# Autodesk Inventor assembly: Drive Roller Assembly 2
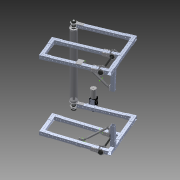
[picture p0: Inventor's stored thumbnail of the model, 180x180]
Saved by Autodesk Inventor 2014 (Build 180170000, 170)
## iProperties
Created: 2014-01-12
Part Number: Drive Roller Assembly 2
Document SubType Name: Assembly
Designer: Michael
Mass: 4500.32 g
Surface Area: 14923 cm^2
Volume: 1330.27 cm^3
Density: 3.383 g/cm^3
Author: Michael
## Documents named in this file (23)
- C:\Users\Michael\Documents\GitHub\2014buildCAD\New Collector\Drive Roller Assembly 2.iam
- C:\Users\Michael\Documents\GitHub\2014buildCAD\Collector\Hex Shaft Collar 1-2 in (7552K500).ipt
- C:\Users\Michael\Documents\GitHub\2014buildCAD\Collector\Roller End Cap Drive (3-D Printed).ipt
- C:\Users\Michael\Documents\GitHub\2014buildCAD\Collector\Vex Pro VersaPlanetary Side Mount.ipt
- C:\Users\Michael\Documents\GitHub\2014buildCAD\Collector\VersaPlanetary (Fixed).iam
- C:\Users\Michael\Documents\GitHub\2014buildCAD\New Collector\Polycarbonate Roller 2 OD 1-16 Thick (8585K64).ipt
- C:\Users\Michael\Documents\GitHub\2014buildCAD\New Collector\Hex Bearing 1-2 in (FR8ZZ-Hex, am-0279).ipt
- C:\Users\Michael\Documents\GitHub\2014buildCAD\New Collector\Hex Shaft Collar 1-2 in (7552K500).ipt
- C:\Users\Michael\Documents\GitHub\2014buildCAD\New Collector\Roller End Cap Drive (3-D Printed).ipt
- C:\Users\Michael\Documents\GitHub\2014buildCAD\New Collector\Vex Pro End Bearing Mount.ipt
- C:\Users\Michael\Documents\GitHub\2014buildCAD\New Collector\Vex Pro 1x1 rectangular tubing 14 in length.ipt
- C:\Users\Michael\Documents\GitHub\2014buildCAD\New Collector\Hex Shaft Aluminum 1-2 in (am-2291).ipt
- C:\Users\Michael\Documents\GitHub\2014buildCAD\New Collector\Timing Pulley (HTD 5mm) - 18T 9mm Double Flange, 1-2 in Hex (VexPro).ipt
- C:\Users\Michael\Documents\GitHub\2014buildCAD\New Collector\Clamp with Piston Assembly.iam
- C:\Users\Michael\Documents\GitHub\2014buildCAD\New Collector\Vex Pro 90 degree gusset.ipt
- C:\Users\Michael\Documents\GitHub\2014buildCAD\New Collector\Vex Pro 1x1 rectangular tubing 2 in length.ipt
- C:\Users\Michael\Documents\GitHub\2014buildCAD\New Collector\Hex Shaft 3-8 in (am-0855).ipt
- C:\Users\Michael\Documents\GitHub\2014buildCAD\New Collector\Hex Shaft Collar 3-8 in (7552K300).ipt
- C:\Users\Michael\Documents\GitHub\2014buildCAD\New Collector\3 Postion Pneumatic Cylinder (9-16 in Bore, .25 in,2 in stroke).iam
- C:\Users\Michael\Documents\GitHub\2014buildCAD\New Collector\Vex Pro 1x1 rectangular tubing 6 in length.ipt
- C:\Users\Michael\Documents\GitHub\2014buildCAD\New Collector\Pneumatic Piston Back Flange (Custom).ipt
- C:\Users\Michael\Documents\GitHub\2014buildCAD\New Collector\Pneumatic Piston Front Flange (Custom).ipt
- C:\Users\Michael\Documents\GitHub\2014buildCAD\New Collector\Pneumatic Piston Front Flange (Right Custom).ipt
## Components (61 placed, 20 different names)
1. Roller End Cap Drive (3-D Printed):2 — Mate:154, Mate:155, Mate:156, Mate:157, Mate:158
2. Vex Pro VersaPlanetary Side Mount:1 — Insert:29, Insert:30, Mate:136, Mate:181, Mate:182
3. VersaPlanetary (Fixed):1 [sub-assembly] — Insert:29, Insert:30, Mate:113, Mate:114, Mate:120, Mate:121, Mate:153
4. Hex Shaft Collar 1-2 in (7552K500):9 — Mate:113, Mate:114
5. Hex Shaft Collar 1-2 in (7552K500):10 — Mate:120, Mate:121
6. Polycarbonate Roller 2 OD 1-16 Thick (8585K64):3 — Mate:157, Mate:158, Mate:159, Mate:160
7. Hex Bearing 1-2 in (FR8ZZ-Hex, am-0279):3 — Mate:128, Mate:129, Mate:134, Mate:156
8. Roller End Cap Drive (3-D Printed):5 — Mate:159, Mate:160, Mate:174
9. Vex Pro 1x1 rectangular tubing 14 in length:2 — Mate:122, Mate:123, Mate:124, Mate:125, Mate:126, Mate:127, Mate:136, Mate:181, Mate:182, Mate:198, Mate:199, Mate:200, Flush:9
10. Hex Shaft Aluminum 1-2 in (am-2291):1 — Flush:1, Mate:132, Mate:133, Mate:134, Mate:143, Mate:144, Mate:146, Mate:147, Mate:154, Mate:155, Mate:172, Mate:173, Mate:175, Mate:176, Mate:179, Mate:180
11. Vex Pro End Bearing Mount:4 — Mate:122, Mate:123, Mate:126, Mate:130, Mate:131
12. Vex Pro End Bearing Mount:5 — Mate:124, Mate:125, Mate:127, Mate:128, Mate:129
13. Hex Bearing 1-2 in (FR8ZZ-Hex, am-0279):4 — Mate:130, Mate:131, Flush:1, Mate:132, Mate:133, Mate:161
14. Timing Pulley (HTD 5mm) - 18T 9mm Double Flange, 1-2 in Hex (VexPro):3 — Mate:143, Mate:144, Mate:145, Mate:161
15. Hex Shaft Collar 1-2 in (7552K500):13 — Mate:145, Mate:146, Mate:147, Flush:2
16. Hex Shaft Collar 1-2 in (7552K500):14 — Flush:4, Mate:152
17. Timing Pulley (HTD 5mm) - 18T 9mm Double Flange, 1-2 in Hex (VexPro):4 — Mate:150, Flush:3, Mate:151, Flush:4, Mate:152
18. Hex Shaft Collar 1-2 in (7552K500):15 — Flush:2, Mate:150, Flush:3, Mate:151, Mate:153
19. Hex Bearing 1-2 in (FR8ZZ-Hex, am-0279):5 — Mate:178
20. Vex Pro 1x1 rectangular tubing 14 in length:3 — Mate:183, Mate:184, Mate:185, Mate:186, Mate:187, Mate:188, Flush:9
21. Vex Pro End Bearing Mount:7
22. Vex Pro End Bearing Mount:8
23. Hex Bearing 1-2 in (FR8ZZ-Hex, am-0279):6 — Mate:172, Mate:173, Mate:177
24. Hex Shaft Collar 1-2 in (7552K500):16 — Mate:178, Mate:179, Mate:180
25. Hex Shaft Collar 1-2 in (7552K500):17 — Mate:174, Mate:175, Mate:176, Mate:177
26. Clamp with Piston Assembly:1 [sub-assembly] — Mate:226, Mate:227, Flush:6, Mate:230, Mate:233, Mate:285, Mate:286, Mate:287
27. Vex Pro 1x1 rectangular tubing 14 in length:5 — Mate:189, Mate:190, Mate:191, Mate:203, Mate:210, Mate:211, Mate:221, Mate:222, Mate:223, Mate:264, Mate:265, Mate:266, Mate:267, Mate:268, Mate:269, Mate:270, Mate:272, Mate:273
28. Vex Pro 90 degree gusset:1 — Mate:186, Mate:187, Mate:188
29. Vex Pro 90 degree gusset:3 — Mate:183, Mate:184, Mate:185, Mate:189, Mate:190, Mate:191
30. Vex Pro 1x1 rectangular tubing 14 in length:6 — Mate:195, Mate:196, Mate:197, Mate:258, Mate:259, Mate:260, Mate:261, Mate:262, Mate:263, Mate:298, Mate:299, Mate:300, Mate:301, Mate:305, Mate:306
31. Vex Pro 90 degree gusset:5 — Mate:195, Mate:196, Mate:197, Mate:198, Mate:199, Mate:200
32. Vex Pro 90 degree gusset:6
33. Vex Pro 90 degree gusset:8 — Mate:203, Mate:210, Mate:211, Mate:212, Mate:213, Mate:214
34. Vex Pro 1x1 rectangular tubing 2 in length:1 — Mate:212, Mate:213, Mate:214
35. Vex Pro 90 degree gusset:10 — Mate:221, Mate:222, Mate:223
36. Vex Pro 1x1 rectangular tubing 2 in length:2 — Mate:224, Mate:225, Flush:5, Mate:271
37. Hex Shaft 3-8 in (am-0855):1 — Mate:224, Mate:225, Flush:5, Mate:226, Mate:227, Flush:6, Mate:228, Mate:229, Mate:231, Mate:232
38. Hex Shaft Collar 3-8 in (7552K300):1 — Mate:228, Mate:229, Mate:230
39. Hex Shaft Collar 3-8 in (7552K300):2 — Mate:231, Mate:232, Mate:233
40. Clamp with Piston Assembly:2 [sub-assembly] — Mate:311, Mate:312, Mate:313
41. Vex Pro 90 degree gusset:11 — Mate:253, Mate:254, Mate:255
42. Vex Pro 90 degree gusset:12 — Mate:261, Mate:262, Mate:263
43. Vex Pro 1x1 rectangular tubing 2 in length:3 — Mate:253, Mate:254, Mate:255
44. Vex Pro 90 degree gusset:13 — Mate:258, Mate:259, Mate:260
45. Vex Pro 1x1 rectangular tubing 2 in length:4
46. Hex Shaft 3-8 in (am-0855):2
47. Hex Shaft Collar 3-8 in (7552K300):3
48. Hex Shaft Collar 3-8 in (7552K300):4
49. 3 Postion Pneumatic Cylinder (9-16 in Bore, .25 in,2 in stroke):1 [sub-assembly] — Mate:280, Mate:281, Mate:282, Mate:288
50. Vex Pro 1x1 rectangular tubing 6 in length:1 — Mate:274, Mate:275, Mate:276, Mate:277, Mate:278, Mate:279
51. Vex Pro 90 degree gusset:14 — Mate:264, Mate:265, Mate:266, Mate:274, Mate:275, Mate:276
52. Vex Pro 90 degree gusset:15 — Mate:267, Mate:268, Mate:269
53. Vex Pro 90 degree gusset:16 — Mate:270, Mate:271, Mate:272, Mate:273
54. Pneumatic Piston Back Flange (Custom):1 — Mate:277, Mate:278, Mate:279, Mate:280, Mate:281, Mate:282
55. Pneumatic Piston Front Flange (Custom):1 — Mate:285, Mate:286, Mate:287, Mate:288
56. 3 Postion Pneumatic Cylinder (9-16 in Bore, .25 in,2 in stroke):2 [sub-assembly] — Mate:314
57. Vex Pro 1x1 rectangular tubing 6 in length:2 — Mate:302, Mate:303, Mate:304, Mate:307, Mate:308
58. Vex Pro 90 degree gusset:17 — Mate:300, Mate:301, Mate:305, Mate:306
59. Vex Pro 90 degree gusset:18 — Mate:298, Mate:299, Mate:302, Mate:303, Mate:304
60. Pneumatic Piston Back Flange (Custom):2 — Mate:307, Mate:308
61. Pneumatic Piston Front Flange (Right Custom):1 — Mate:311, Mate:312, Mate:313, Mate:314
## Relationships (177: Mate 166, Flush 9, Insert 2)
- Insert:29: Vex Pro VersaPlanetary Side Mount:1 ↔ VersaPlanetary (Fixed):1
- Insert:30: Vex Pro VersaPlanetary Side Mount:1 ↔ VersaPlanetary (Fixed):1
- Mate:113: VersaPlanetary (Fixed):1 ↔ Hex Shaft Collar 1-2 in (7552K500):9
- Mate:114: VersaPlanetary (Fixed):1 ↔ Hex Shaft Collar 1-2 in (7552K500):9
- Mate:120: VersaPlanetary (Fixed):1 ↔ Hex Shaft Collar 1-2 in (7552K500):10
- Mate:121: VersaPlanetary (Fixed):1 ↔ Hex Shaft Collar 1-2 in (7552K500):10
- Mate:122: Vex Pro 1x1 rectangular tubing 14 in length:2 ↔ Vex Pro End Bearing Mount:4
- Mate:123: Vex Pro 1x1 rectangular tubing 14 in length:2 ↔ Vex Pro End Bearing Mount:4
- Mate:124: Vex Pro 1x1 rectangular tubing 14 in length:2 ↔ Vex Pro End Bearing Mount:5
- Mate:125: Vex Pro 1x1 rectangular tubing 14 in length:2 ↔ Vex Pro End Bearing Mount:5
- Mate:126: Vex Pro 1x1 rectangular tubing 14 in length:2 ↔ Vex Pro End Bearing Mount:4
- Mate:127: Vex Pro 1x1 rectangular tubing 14 in length:2 ↔ Vex Pro End Bearing Mount:5
- Mate:128: Hex Bearing 1-2 in (FR8ZZ-Hex, am-0279):3 ↔ Vex Pro End Bearing Mount:5
- Mate:129: Hex Bearing 1-2 in (FR8ZZ-Hex, am-0279):3 ↔ Vex Pro End Bearing Mount:5
- Mate:130: Vex Pro End Bearing Mount:4 ↔ Hex Bearing 1-2 in (FR8ZZ-Hex, am-0279):4
- Mate:131: Vex Pro End Bearing Mount:4 ↔ Hex Bearing 1-2 in (FR8ZZ-Hex, am-0279):4
- Flush:1 (-25.4 mm): Hex Shaft Aluminum 1-2 in (am-2291):1 ↔ Hex Bearing 1-2 in (FR8ZZ-Hex, am-0279):4
- Mate:132: Hex Shaft Aluminum 1-2 in (am-2291):1 ↔ Hex Bearing 1-2 in (FR8ZZ-Hex, am-0279):4
- Mate:133: Hex Shaft Aluminum 1-2 in (am-2291):1 ↔ Hex Bearing 1-2 in (FR8ZZ-Hex, am-0279):4
- Mate:134: Hex Bearing 1-2 in (FR8ZZ-Hex, am-0279):3 ↔ Hex Shaft Aluminum 1-2 in (am-2291):1
- Mate:136: Vex Pro VersaPlanetary Side Mount:1 ↔ Vex Pro 1x1 rectangular tubing 14 in length:2
- Mate:143: Hex Shaft Aluminum 1-2 in (am-2291):1 ↔ Timing Pulley (HTD 5mm) - 18T 9mm Double Flange, 1-2 in Hex (VexPro):3
- Mate:144: Hex Shaft Aluminum 1-2 in (am-2291):1 ↔ Timing Pulley (HTD 5mm) - 18T 9mm Double Flange, 1-2 in Hex (VexPro):3
- Mate:145: Timing Pulley (HTD 5mm) - 18T 9mm Double Flange, 1-2 in Hex (VexPro):3 ↔ Hex Shaft Collar 1-2 in (7552K500):13
- Mate:146: Hex Shaft Aluminum 1-2 in (am-2291):1 ↔ Hex Shaft Collar 1-2 in (7552K500):13
- Mate:147: Hex Shaft Aluminum 1-2 in (am-2291):1 ↔ Hex Shaft Collar 1-2 in (7552K500):13
- [Mate]: Hex Shaft Collar 1-2 in (7552K500):14 ↔ Timing Pulley (HTD 5mm) - 18T 9mm Double Flange, 1-2 in Hex (VexPro):4
- [Mate]: Timing Pulley (HTD 5mm) - 18T 9mm Double Flange, 1-2 in Hex (VexPro):4 ↔ Hex Shaft Collar 1-2 in (7552K500):15
- Flush:2: Hex Shaft Collar 1-2 in (7552K500):13 ↔ Hex Shaft Collar 1-2 in (7552K500):15
- Mate:150: Timing Pulley (HTD 5mm) - 18T 9mm Double Flange, 1-2 in Hex (VexPro):4 ↔ Hex Shaft Collar 1-2 in (7552K500):15
- Flush:3: Timing Pulley (HTD 5mm) - 18T 9mm Double Flange, 1-2 in Hex (VexPro):4 ↔ Hex Shaft Collar 1-2 in (7552K500):15
- Mate:151: Timing Pulley (HTD 5mm) - 18T 9mm Double Flange, 1-2 in Hex (VexPro):4 ↔ Hex Shaft Collar 1-2 in (7552K500):15
- Flush:4: Hex Shaft Collar 1-2 in (7552K500):14 ↔ Timing Pulley (HTD 5mm) - 18T 9mm Double Flange, 1-2 in Hex (VexPro):4
- Mate:152: Hex Shaft Collar 1-2 in (7552K500):14 ↔ Timing Pulley (HTD 5mm) - 18T 9mm Double Flange, 1-2 in Hex (VexPro):4
- Mate:153: VersaPlanetary (Fixed):1 ↔ Hex Shaft Collar 1-2 in (7552K500):15
- Mate:154: Roller End Cap Drive (3-D Printed):2 ↔ Hex Shaft Aluminum 1-2 in (am-2291):1
- Mate:155: Roller End Cap Drive (3-D Printed):2 ↔ Hex Shaft Aluminum 1-2 in (am-2291):1
- Mate:156: Roller End Cap Drive (3-D Printed):2 ↔ Hex Bearing 1-2 in (FR8ZZ-Hex, am-0279):3
- Mate:157: Roller End Cap Drive (3-D Printed):2 ↔ Polycarbonate Roller 2 OD 1-16 Thick (8585K64):3
- Mate:158: Roller End Cap Drive (3-D Printed):2 ↔ Polycarbonate Roller 2 OD 1-16 Thick (8585K64):3
- Mate:159: Polycarbonate Roller 2 OD 1-16 Thick (8585K64):3 ↔ Roller End Cap Drive (3-D Printed):5
- Mate:160: Polycarbonate Roller 2 OD 1-16 Thick (8585K64):3 ↔ Roller End Cap Drive (3-D Printed):5
- Mate:161: Hex Bearing 1-2 in (FR8ZZ-Hex, am-0279):4 ↔ Timing Pulley (HTD 5mm) - 18T 9mm Double Flange, 1-2 in Hex (VexPro):3
- [Mate]: Vex Pro 1x1 rectangular tubing 14 in length:3 ↔ Vex Pro End Bearing Mount:7
- [Mate]: Vex Pro 1x1 rectangular tubing 14 in length:3 ↔ Vex Pro End Bearing Mount:7
- [Mate]: Vex Pro 1x1 rectangular tubing 14 in length:3 ↔ Vex Pro End Bearing Mount:8
- [Mate]: Vex Pro 1x1 rectangular tubing 14 in length:3 ↔ Vex Pro End Bearing Mount:8
- [Mate]: Vex Pro 1x1 rectangular tubing 14 in length:3 ↔ Vex Pro End Bearing Mount:7
- [Mate]: Vex Pro 1x1 rectangular tubing 14 in length:3 ↔ Vex Pro End Bearing Mount:8
- [Mate]: Hex Bearing 1-2 in (FR8ZZ-Hex, am-0279):5 ↔ Vex Pro End Bearing Mount:8
- [Mate]: Hex Bearing 1-2 in (FR8ZZ-Hex, am-0279):5 ↔ Vex Pro End Bearing Mount:8
- [Mate]: Vex Pro End Bearing Mount:7 ↔ Hex Bearing 1-2 in (FR8ZZ-Hex, am-0279):6
- [Mate]: Vex Pro End Bearing Mount:7 ↔ Hex Bearing 1-2 in (FR8ZZ-Hex, am-0279):6
- Mate:172: Hex Shaft Aluminum 1-2 in (am-2291):1 ↔ Hex Bearing 1-2 in (FR8ZZ-Hex, am-0279):6
- Mate:173: Hex Shaft Aluminum 1-2 in (am-2291):1 ↔ Hex Bearing 1-2 in (FR8ZZ-Hex, am-0279):6
- Mate:174: Roller End Cap Drive (3-D Printed):5 ↔ Hex Shaft Collar 1-2 in (7552K500):17
- Mate:175: Hex Shaft Aluminum 1-2 in (am-2291):1 ↔ Hex Shaft Collar 1-2 in (7552K500):17
- Mate:176: Hex Shaft Aluminum 1-2 in (am-2291):1 ↔ Hex Shaft Collar 1-2 in (7552K500):17
- Mate:177: Hex Bearing 1-2 in (FR8ZZ-Hex, am-0279):6 ↔ Hex Shaft Collar 1-2 in (7552K500):17
- Mate:178: Hex Bearing 1-2 in (FR8ZZ-Hex, am-0279):5 ↔ Hex Shaft Collar 1-2 in (7552K500):16
- Mate:179: Hex Shaft Aluminum 1-2 in (am-2291):1 ↔ Hex Shaft Collar 1-2 in (7552K500):16
- Mate:180: Hex Shaft Aluminum 1-2 in (am-2291):1 ↔ Hex Shaft Collar 1-2 in (7552K500):16
- Mate:181: Vex Pro VersaPlanetary Side Mount:1 ↔ Vex Pro 1x1 rectangular tubing 14 in length:2
- Mate:182: Vex Pro VersaPlanetary Side Mount:1 ↔ Vex Pro 1x1 rectangular tubing 14 in length:2
- Mate:183: Vex Pro 1x1 rectangular tubing 14 in length:3 ↔ Vex Pro 90 degree gusset:3
- Mate:184: Vex Pro 1x1 rectangular tubing 14 in length:3 ↔ Vex Pro 90 degree gusset:3
- Mate:185: Vex Pro 1x1 rectangular tubing 14 in length:3 ↔ Vex Pro 90 degree gusset:3
- Mate:186: Vex Pro 1x1 rectangular tubing 14 in length:3 ↔ Vex Pro 90 degree gusset:1
- Mate:187: Vex Pro 1x1 rectangular tubing 14 in length:3 ↔ Vex Pro 90 degree gusset:1
- Mate:188: Vex Pro 1x1 rectangular tubing 14 in length:3 ↔ Vex Pro 90 degree gusset:1
- Mate:189: Vex Pro 1x1 rectangular tubing 14 in length:5 ↔ Vex Pro 90 degree gusset:3
- Mate:190: Vex Pro 1x1 rectangular tubing 14 in length:5 ↔ Vex Pro 90 degree gusset:3
- Mate:191: Vex Pro 1x1 rectangular tubing 14 in length:5 ↔ Vex Pro 90 degree gusset:3
- [Mate]: Vex Pro 1x1 rectangular tubing 14 in length:6 ↔ Vex Pro 90 degree gusset:6
- [Mate]: Vex Pro 1x1 rectangular tubing 14 in length:6 ↔ Vex Pro 90 degree gusset:6
- [Mate]: Vex Pro 1x1 rectangular tubing 14 in length:6 ↔ Vex Pro 90 degree gusset:6
- Mate:195: Vex Pro 1x1 rectangular tubing 14 in length:6 ↔ Vex Pro 90 degree gusset:5
- Mate:196: Vex Pro 1x1 rectangular tubing 14 in length:6 ↔ Vex Pro 90 degree gusset:5
- Mate:197: Vex Pro 1x1 rectangular tubing 14 in length:6 ↔ Vex Pro 90 degree gusset:5
- Mate:198: Vex Pro 1x1 rectangular tubing 14 in length:2 ↔ Vex Pro 90 degree gusset:5
- Mate:199: Vex Pro 1x1 rectangular tubing 14 in length:2 ↔ Vex Pro 90 degree gusset:5
- Mate:200: Vex Pro 1x1 rectangular tubing 14 in length:2 ↔ Vex Pro 90 degree gusset:5
- Mate:203: Vex Pro 1x1 rectangular tubing 14 in length:5 ↔ Vex Pro 90 degree gusset:8
- Mate:210: Vex Pro 1x1 rectangular tubing 14 in length:5 ↔ Vex Pro 90 degree gusset:8
- Mate:211: Vex Pro 1x1 rectangular tubing 14 in length:5 ↔ Vex Pro 90 degree gusset:8
- Mate:212: Vex Pro 90 degree gusset:8 ↔ Vex Pro 1x1 rectangular tubing 2 in length:1
- Mate:213: Vex Pro 90 degree gusset:8 ↔ Vex Pro 1x1 rectangular tubing 2 in length:1
- Mate:214: Vex Pro 90 degree gusset:8 ↔ Vex Pro 1x1 rectangular tubing 2 in length:1
- [Mate]: Vex Pro 90 degree gusset:10 ↔ Vex Pro 1x1 rectangular tubing 2 in length:2
- [Mate]: Vex Pro 90 degree gusset:10 ↔ Vex Pro 1x1 rectangular tubing 2 in length:2
- [Mate]: Vex Pro 90 degree gusset:10 ↔ Vex Pro 1x1 rectangular tubing 2 in length:2
- Mate:221: Vex Pro 1x1 rectangular tubing 14 in length:5 ↔ Vex Pro 90 degree gusset:10
- Mate:222: Vex Pro 1x1 rectangular tubing 14 in length:5 ↔ Vex Pro 90 degree gusset:10
- Mate:223: Vex Pro 1x1 rectangular tubing 14 in length:5 ↔ Vex Pro 90 degree gusset:10
- Mate:224: Vex Pro 1x1 rectangular tubing 2 in length:2 ↔ Hex Shaft 3-8 in (am-0855):1
- Mate:225: Vex Pro 1x1 rectangular tubing 2 in length:2 ↔ Hex Shaft 3-8 in (am-0855):1
- Flush:5 (-19.05 mm): Vex Pro 1x1 rectangular tubing 2 in length:2 ↔ Hex Shaft 3-8 in (am-0855):1
- Mate:226: Clamp with Piston Assembly:1 ↔ Hex Shaft 3-8 in (am-0855):1
- Mate:227: Clamp with Piston Assembly:1 ↔ Hex Shaft 3-8 in (am-0855):1
- Flush:6 (-9.525 mm): Clamp with Piston Assembly:1 ↔ Hex Shaft 3-8 in (am-0855):1
- Mate:228: Hex Shaft 3-8 in (am-0855):1 ↔ Hex Shaft Collar 3-8 in (7552K300):1
- Mate:229: Hex Shaft 3-8 in (am-0855):1 ↔ Hex Shaft Collar 3-8 in (7552K300):1
- Mate:230: Clamp with Piston Assembly:1 ↔ Hex Shaft Collar 3-8 in (7552K300):1
- Mate:231: Hex Shaft 3-8 in (am-0855):1 ↔ Hex Shaft Collar 3-8 in (7552K300):2
- Mate:232: Hex Shaft 3-8 in (am-0855):1 ↔ Hex Shaft Collar 3-8 in (7552K300):2
- Mate:233: Clamp with Piston Assembly:1 ↔ Hex Shaft Collar 3-8 in (7552K300):2
- [Mate]: Vex Pro 90 degree gusset:12 ↔ Vex Pro 1x1 rectangular tubing 2 in length:3
- [Mate]: Vex Pro 90 degree gusset:12 ↔ Vex Pro 1x1 rectangular tubing 2 in length:3
- [Mate]: Vex Pro 90 degree gusset:12 ↔ Vex Pro 1x1 rectangular tubing 2 in length:3
- [Mate]: Vex Pro 90 degree gusset:13 ↔ Vex Pro 1x1 rectangular tubing 2 in length:4
- [Mate]: Vex Pro 90 degree gusset:13 ↔ Vex Pro 1x1 rectangular tubing 2 in length:4
- [Mate]: Vex Pro 90 degree gusset:13 ↔ Vex Pro 1x1 rectangular tubing 2 in length:4
- [Mate]: Vex Pro 1x1 rectangular tubing 2 in length:4 ↔ Hex Shaft 3-8 in (am-0855):2
- [Mate]: Vex Pro 1x1 rectangular tubing 2 in length:4 ↔ Hex Shaft 3-8 in (am-0855):2
- [Flush] (-19.05 mm): Vex Pro 1x1 rectangular tubing 2 in length:4 ↔ Hex Shaft 3-8 in (am-0855):2
- [Mate]: Clamp with Piston Assembly:2 ↔ Hex Shaft 3-8 in (am-0855):2
- [Mate]: Clamp with Piston Assembly:2 ↔ Hex Shaft 3-8 in (am-0855):2
- [Flush] (-9.525 mm): Clamp with Piston Assembly:2 ↔ Hex Shaft 3-8 in (am-0855):2
- [Mate]: Hex Shaft 3-8 in (am-0855):2 ↔ Hex Shaft Collar 3-8 in (7552K300):3
- [Mate]: Hex Shaft 3-8 in (am-0855):2 ↔ Hex Shaft Collar 3-8 in (7552K300):3
- [Mate]: Clamp with Piston Assembly:2 ↔ Hex Shaft Collar 3-8 in (7552K300):3
- [Mate]: Hex Shaft 3-8 in (am-0855):2 ↔ Hex Shaft Collar 3-8 in (7552K300):4
- [Mate]: Hex Shaft 3-8 in (am-0855):2 ↔ Hex Shaft Collar 3-8 in (7552K300):4
- [Mate]: Clamp with Piston Assembly:2 ↔ Hex Shaft Collar 3-8 in (7552K300):4
- Mate:253: Vex Pro 90 degree gusset:11 ↔ Vex Pro 1x1 rectangular tubing 2 in length:3
- Mate:254: Vex Pro 90 degree gusset:11 ↔ Vex Pro 1x1 rectangular tubing 2 in length:3
- Mate:255: Vex Pro 90 degree gusset:11 ↔ Vex Pro 1x1 rectangular tubing 2 in length:3
- Mate:258: Vex Pro 1x1 rectangular tubing 14 in length:6 ↔ Vex Pro 90 degree gusset:13
- Mate:259: Vex Pro 1x1 rectangular tubing 14 in length:6 ↔ Vex Pro 90 degree gusset:13
- Mate:260: Vex Pro 1x1 rectangular tubing 14 in length:6 ↔ Vex Pro 90 degree gusset:13
- Mate:261: Vex Pro 1x1 rectangular tubing 14 in length:6 ↔ Vex Pro 90 degree gusset:12
- Mate:262: Vex Pro 1x1 rectangular tubing 14 in length:6 ↔ Vex Pro 90 degree gusset:12
- Mate:263: Vex Pro 1x1 rectangular tubing 14 in length:6 ↔ Vex Pro 90 degree gusset:12
- Flush:9: Vex Pro 1x1 rectangular tubing 14 in length:2 ↔ Vex Pro 1x1 rectangular tubing 14 in length:3
- Mate:264: Vex Pro 1x1 rectangular tubing 14 in length:5 ↔ Vex Pro 90 degree gusset:14
- Mate:265: Vex Pro 1x1 rectangular tubing 14 in length:5 ↔ Vex Pro 90 degree gusset:14
- Mate:266: Vex Pro 1x1 rectangular tubing 14 in length:5 ↔ Vex Pro 90 degree gusset:14
- Mate:267: Vex Pro 1x1 rectangular tubing 14 in length:5 ↔ Vex Pro 90 degree gusset:15
- Mate:268: Vex Pro 1x1 rectangular tubing 14 in length:5 ↔ Vex Pro 90 degree gusset:15
- Mate:269: Vex Pro 1x1 rectangular tubing 14 in length:5 ↔ Vex Pro 90 degree gusset:15
- Mate:270: Vex Pro 1x1 rectangular tubing 14 in length:5 ↔ Vex Pro 90 degree gusset:16
- Mate:271: Vex Pro 1x1 rectangular tubing 2 in length:2 ↔ Vex Pro 90 degree gusset:16
- Mate:272: Vex Pro 1x1 rectangular tubing 14 in length:5 ↔ Vex Pro 90 degree gusset:16
- Mate:273: Vex Pro 1x1 rectangular tubing 14 in length:5 ↔ Vex Pro 90 degree gusset:16
- Mate:274: Vex Pro 1x1 rectangular tubing 6 in length:1 ↔ Vex Pro 90 degree gusset:14
- Mate:275: Vex Pro 1x1 rectangular tubing 6 in length:1 ↔ Vex Pro 90 degree gusset:14
- Mate:276: Vex Pro 1x1 rectangular tubing 6 in length:1 ↔ Vex Pro 90 degree gusset:14
- Mate:277: Vex Pro 1x1 rectangular tubing 6 in length:1 ↔ Pneumatic Piston Back Flange (Custom):1
- Mate:278: Vex Pro 1x1 rectangular tubing 6 in length:1 ↔ Pneumatic Piston Back Flange (Custom):1
- Mate:279: Vex Pro 1x1 rectangular tubing 6 in length:1 ↔ Pneumatic Piston Back Flange (Custom):1
- Mate:280: 3 Postion Pneumatic Cylinder (9-16 in Bore, .25 in,2 in stroke):1 ↔ Pneumatic Piston Back Flange (Custom):1
- Mate:281: 3 Postion Pneumatic Cylinder (9-16 in Bore, .25 in,2 in stroke):1 ↔ Pneumatic Piston Back Flange (Custom):1
- Mate:282: 3 Postion Pneumatic Cylinder (9-16 in Bore, .25 in,2 in stroke):1 ↔ Pneumatic Piston Back Flange (Custom):1
- Mate:285: Clamp with Piston Assembly:1 ↔ Pneumatic Piston Front Flange (Custom):1
- Mate:286: Clamp with Piston Assembly:1 ↔ Pneumatic Piston Front Flange (Custom):1
- Mate:287: Clamp with Piston Assembly:1 ↔ Pneumatic Piston Front Flange (Custom):1
- Mate:288: 3 Postion Pneumatic Cylinder (9-16 in Bore, .25 in,2 in stroke):1 ↔ Pneumatic Piston Front Flange (Custom):1
- [Mate]: Vex Pro 1x1 rectangular tubing 6 in length:2 ↔ Vex Pro 90 degree gusset:17
- [Mate]: Vex Pro 1x1 rectangular tubing 6 in length:2 ↔ Pneumatic Piston Back Flange (Custom):2
- [Mate]: 3 Postion Pneumatic Cylinder (9-16 in Bore, .25 in,2 in stroke):2 ↔ Pneumatic Piston Back Flange (Custom):2
- [Mate]: 3 Postion Pneumatic Cylinder (9-16 in Bore, .25 in,2 in stroke):2 ↔ Pneumatic Piston Back Flange (Custom):2
- [Mate]: 3 Postion Pneumatic Cylinder (9-16 in Bore, .25 in,2 in stroke):2 ↔ Pneumatic Piston Back Flange (Custom):2
- Mate:298: Vex Pro 1x1 rectangular tubing 14 in length:6 ↔ Vex Pro 90 degree gusset:18
- Mate:299: Vex Pro 1x1 rectangular tubing 14 in length:6 ↔ Vex Pro 90 degree gusset:18
- Mate:300: Vex Pro 1x1 rectangular tubing 14 in length:6 ↔ Vex Pro 90 degree gusset:17
- Mate:301: Vex Pro 1x1 rectangular tubing 14 in length:6 ↔ Vex Pro 90 degree gusset:17
- Mate:302: Vex Pro 1x1 rectangular tubing 6 in length:2 ↔ Vex Pro 90 degree gusset:18
- Mate:303: Vex Pro 1x1 rectangular tubing 6 in length:2 ↔ Vex Pro 90 degree gusset:18
- Mate:304: Vex Pro 1x1 rectangular tubing 6 in length:2 ↔ Vex Pro 90 degree gusset:18
- Mate:305: Vex Pro 1x1 rectangular tubing 14 in length:6 ↔ Vex Pro 90 degree gusset:17
- Mate:306: Vex Pro 1x1 rectangular tubing 14 in length:6 ↔ Vex Pro 90 degree gusset:17
- Mate:307: Vex Pro 1x1 rectangular tubing 6 in length:2 ↔ Pneumatic Piston Back Flange (Custom):2
- Mate:308: Vex Pro 1x1 rectangular tubing 6 in length:2 ↔ Pneumatic Piston Back Flange (Custom):2
- Mate:311: Clamp with Piston Assembly:2 ↔ Pneumatic Piston Front Flange (Right Custom):1
- Mate:312: Clamp with Piston Assembly:2 ↔ Pneumatic Piston Front Flange (Right Custom):1
- Mate:313: Clamp with Piston Assembly:2 ↔ Pneumatic Piston Front Flange (Right Custom):1
- Mate:314: 3 Postion Pneumatic Cylinder (9-16 in Bore, .25 in,2 in stroke):2 ↔ Pneumatic Piston Front Flange (Right Custom):1
## Named parameters: d216_d210 = 0 mm, d217_d213 = 0 mm, d234_d189 = 0 mm, d235_d190 = 0 mm, d236_d191 = 0 mm, d237_d192 = 0 mm, d238_d193 = 0 mm, d239_d194 = 0 mm, d240_d195 = 0 mm, d241_d196 = 0 mm, d242_d197 = 0 mm, d243_d198 = 0 mm, d265_d262 = 0 mm, d266_d263 = 0 mm, d267_d264 = 0 mm, d305_d302 = 0 mm, d306_d303 = 0 mm, d307_d304 = 0 mm, d334_d317 = 0 mm, d335_d318 = -19.05 mm, d336_d325 = 0 mm, d337_d302 = 0 mm, d338_d303 = 0 mm, d339_d304 = 0 mm, d343_d308 = 0 mm, d344_d309 = 0 mm, d345_d310 = 0 mm, d346_d316 = 0 mm, d347_d326 = 0 mm, d348_d327 = -9.525 mm, d349_d328 = 0 mm, d350_d329 = 0 mm, d351_d330 = 0 mm, d352_d331 = 0 mm, d353_d332 = 0 mm, d354_d333 = 0 mm, d399_d379 = 0 mm, d402_d382 = 0 mm, d403_d383 = 0 mm, d404_d384 = 0 mm, d405_d385 = 0 mm
